# Autodesk Inventor assembly: Boitier + PCB
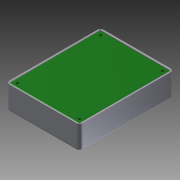
[picture p0: Inventor's stored thumbnail of the model, 180x180]
Saved by Autodesk Inventor 2013 (Build 170138000, 138)
## iProperties
Created: 2013-04-17
Part Number: Boitier + PCB
Document SubType Name: Assembly
Designer: dimercur
Author: dimercur
## Documents named in this file (3)
- U:\Altium\Ada4Arm\Meca\Boitier + PCB.iam
- U:\Altium\Ada4Arm\Meca\boitier.iam
- U:\Altium\Ada4Arm\Meca\pcb.ipt
## Components (2 placed, 2 different names)
1. boitier:1 [sub-assembly] — Placage:1, Placage:2, Placage:3
2. pcb:1 — Placage:1, Placage:2, Placage:3
## Relationships (3: Mate 3)
- Placage:1 [Mate]: boitier:1 ↔ pcb:1
- Placage:2 [Mate]: boitier:1 ↔ pcb:1
- Placage:3 [Mate] (0.1 mm): boitier:1 ↔ pcb:1
